# Autodesk Inventor assembly: сборка блока аккумуляторов
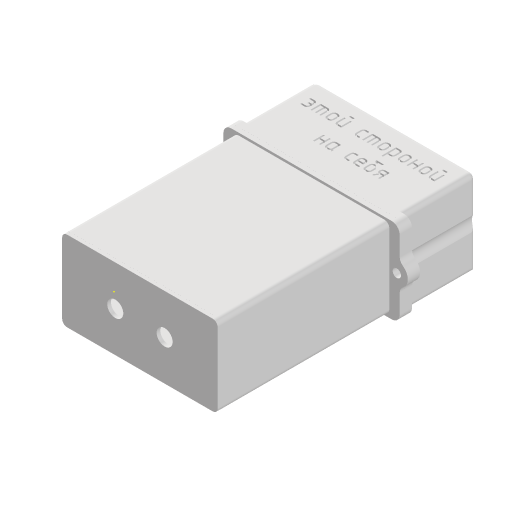
[picture p0: Inventor's stored thumbnail of the model, 512x512]
Saved by Autodesk Inventor 2023.2 (Build 272271000, 271)
## iProperties
Created: 2023-03-03
Part Number: сборка блока аккумуляторов
Document SubType Name: Assembly
Designer: User
Author: User
## Documents named in this file (4)
- C:\Users\matvey\Desktop\YandexDisk\облачное хранилище\НАСУ\Inventor\сборка блока аккумуляторов.iam
- C:\Users\matvey\Desktop\YandexDisk\облачное хранилище\НАСУ\Inventor\нижняя часть блока аккумов.ipt
- C:\Users\matvey\Desktop\YandexDisk\облачное хранилище\НАСУ\Inventor\нижняя часть держателя аккумов.ipt
- C:\Users\matvey\Desktop\YandexDisk\облачное хранилище\НАСУ\Inventor\верхняя часть держателя аккумулятора.ipt
## Components (3 placed, 3 different names)
1. нижняя часть блока аккумов:1 — Совмещение:1, Совмещение:2, Совмещение:3
2. нижняя часть держателя аккумов:1 — Совмещение:1, Совмещение:2, Совмещение:3, Совмещение:4, Совмещение:5, Совмещение:6
3. верхняя часть держателя аккумулятора:1 — Совмещение:4, Совмещение:5, Совмещение:6
## Relationships (6: Mate 6)
- Совмещение:1 [Mate]: нижняя часть блока аккумов:1 ↔ нижняя часть держателя аккумов:1
- Совмещение:2 [Mate]: нижняя часть блока аккумов:1 ↔ нижняя часть держателя аккумов:1
- Совмещение:3 [Mate]: нижняя часть блока аккумов:1 ↔ нижняя часть держателя аккумов:1
- Совмещение:4 [Mate]: нижняя часть держателя аккумов:1 ↔ верхняя часть держателя аккумулятора:1
- Совмещение:5 [Mate]: нижняя часть держателя аккумов:1 ↔ верхняя часть держателя аккумулятора:1
- Совмещение:6 [Mate]: нижняя часть держателя аккумов:1 ↔ верхняя часть держателя аккумулятора:1
